# Autodesk Inventor assembly: JR3_sensor_setup
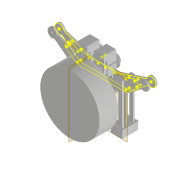
[picture p0: Inventor's stored thumbnail of the model, 180x180]
Saved by Autodesk Inventor 2022 (Build 260153000, 153)
## iProperties
Created: 2022-12-25
Part Number: JR3_sensor_setup
Document SubType Name: Assembly
Designer: dell
Author: dell
## Documents named in this file (4)
- D:\xxxx\Uni\Part IV\MECHENG_700\Part_IV_project_CAD\Bird_skeleton_prototypes\Wing_drone_V1\JR3_sensor_setup\JR3_sensor_setup.iam
- D:\xxxx\Uni\Part IV\MECHENG_700\Part_IV_project_CAD\Bird_skeleton_prototypes\Wing_drone_V1\JR3_sensor_setup\JR3_sensor.ipt
- D:\xxxx\Uni\Part IV\MECHENG_700\Part_IV_project_CAD\Bird_skeleton_prototypes\Wing_drone_V1\Bird_wing_V2\Wing_shoulder\Shoulder_support_assembly.iam
- D:\xxxx\Uni\Part IV\MECHENG_700\Part_IV_project_CAD\Bird_skeleton_prototypes\Wing_drone_V1\JR3_sensor_setup\Plate_0.ipt
## Components (3 placed, 3 different names)
1. JR3_sensor:1 — Mate:1, Mate:2, Mate:3, Mate:4
2. Shoulder_support_assembly:2 [sub-assembly] — Mate:1, Mate:5, Mate:6
3. Plate_0:1 — Mate:2, Mate:3, Mate:4, Mate:5, Mate:6
## Relationships (6: Mate 6)
- Mate:1: JR3_sensor:1 ↔ Shoulder_support_assembly:2
- Mate:2: JR3_sensor:1 ↔ Plate_0:1
- Mate:3: JR3_sensor:1 ↔ Plate_0:1
- Mate:4: JR3_sensor:1 ↔ Plate_0:1
- Mate:5: Shoulder_support_assembly:2 ↔ Plate_0:1
- Mate:6: Shoulder_support_assembly:2 ↔ Plate_0:1
